# Autodesk Inventor assembly: Assembly1
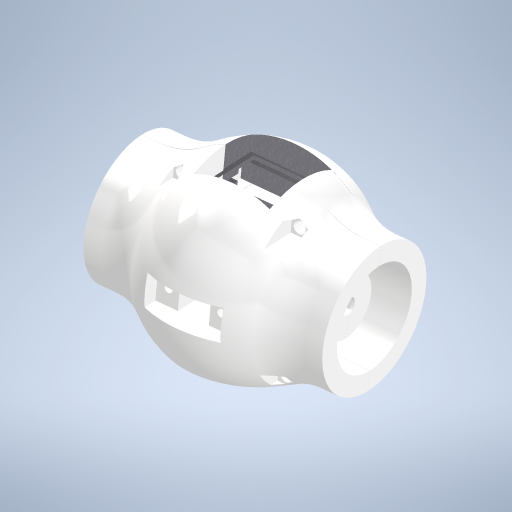
[picture p0: Inventor's stored thumbnail of the model, 512x512]
Saved by Autodesk Inventor 2023 (Build 270158000, 158)
## iProperties
Created: 2022-12-16
Part Number: Assembly1
Document SubType Name: Assembly
Designer: ellie
Author: ellie
## Documents named in this file (4)
- C:\Users\RM206user\Desktop\cansat\tanekonsat2022_runback\machinary\parts\tale\Assembly1.iam
- C:\Users\RM206user\Desktop\cansat\tanekonsat2022_runback\machinary\body\body back\back moter middle tire ver\back moter lemon tale.ipt
- C:\Users\RM206user\Desktop\cansat\tanekonsat2022_runback\machinary\body\body back\back moter middle tire ver\back back gabagaba.ipt
- C:\Users\RM206user\Desktop\cansat\tanekonsat2022_runback\machinary\body\body front\front moter middle basic\body front moter middle lemon shape for printing.ipt
## Components (3 placed, 2 different names)
1. body moter middle:1 — フラッシュ:1, メイト:3, メイト:4, メイト:5, フラッシュ:2, メイト:6
2. body moter middle:2 — フラッシュ:1, メイト:3, メイト:4
3. base front:1 — メイト:5, フラッシュ:2, メイト:6
## Relationships (6: Mate 4, Flush 2)
- フラッシュ:1 [Flush]: body moter middle:1 ↔ body moter middle:2
- メイト:3 [Mate]: body moter middle:1 ↔ body moter middle:2
- メイト:4 [Mate] (0.5 mm): body moter middle:1 ↔ body moter middle:2
- メイト:5 [Mate]: body moter middle:1 ↔ base front:1
- フラッシュ:2 [Flush]: body moter middle:1 ↔ base front:1
- メイト:6 [Mate]: body moter middle:1 ↔ base front:1
